# Autodesk Inventor assembly: HopperAssembly
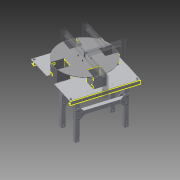
[picture p0: Inventor's stored thumbnail of the model, 180x180]
Saved by Autodesk Inventor 2013 (Build 170138000, 138)
## iProperties
Created: 2013-07-18
Part Number: HopperAssembly
Document SubType Name: Assembly
Designer: root
Author: root
## Documents named in this file (20)
- I:\FRC_Projects\Cad\Inventor_Projects\Shooter-Cleaned\HopperAssembly\HopperAssembly.iam
- I:\FRC_Projects\Cad\Inventor_Projects\Shooter-Cleaned\HopperAssembly\TopHopper\TopHopper.iam
- I:\FRC_Projects\Cad\Inventor_Projects\Shooter-Cleaned\HopperAssembly\BottomHopper\BottomHopperAssembly.iam
- I:\FRC_Projects\Cad\Inventor_Projects\Shooter-Cleaned\HopperAssembly\CouplerBridge.ipt
- I:\FRC_Projects\Cad\Inventor_Projects\Shooter-Cleaned\Libraries\ContentCenter\ANSI_ASME B18.2.1 - 1_4-20 UNC - 0.75(2).ipt
- I:\FRC_Projects\Cad\Inventor_Projects\Shooter-Cleaned\Libraries\ContentCenter\AS 2465 - 1_4  UNC(1).ipt
- I:\FRC_Projects\Cad\Inventor_Projects\Shooter-Cleaned\HopperAssembly\SpacerPvc.ipt
- I:\FRC_Projects\Cad\Inventor_Projects\Shooter-Cleaned\Libraries\ContentCenter\ANSI B18.2.2 - 1_4 - 20(2).ipt
- I:\FRC_Projects\Cad\Inventor_Projects\Shooter-Cleaned\HopperAssembly\BottomSupportBAse.ipt
- I:\FRC_Projects\Cad\Inventor_Projects\Shooter-Cleaned\HopperAssembly\BackBottonSupport.ipt
- I:\FRC_Projects\Cad\Inventor_Projects\Shooter-Cleaned\HopperAssembly\L-Bracket.ipt
- I:\FRC_Projects\Cad\Inventor_Projects\Shooter-Cleaned\Libraries\ContentCenter\ANSI_ASME B18.2.1 - 1_4-20 UNC - 1.5(2).ipt
- I:\FRC_Projects\Cad\Inventor_Projects\Shooter-Cleaned\Libraries\ContentCenter\ANSI_ASME B18.2.1 - 1_4-20 UNC - 1.75(2).ipt
- I:\FRC_Projects\Cad\Inventor_Projects\Shooter-Cleaned\HopperAssembly\TriangleBracket.ipt
- I:\FRC_Projects\Cad\Inventor_Projects\Shooter-Cleaned\HopperAssembly\BAseBAr.ipt
- I:\FRC_Projects\Cad\Inventor_Projects\Shooter-Cleaned\HopperAssembly\CrossBar.ipt
- I:\FRC_Projects\Cad\Inventor_Projects\Shooter-Cleaned\HopperAssembly\SupportT.ipt
- I:\FRC_Projects\Cad\Inventor_Projects\Shooter-Cleaned\Libraries\ContentCenter\ANSI B18.6.3 - 1_4-20 UNC - 3.25(30).ipt
- I:\FRC_Projects\Cad\Inventor_Projects\Shooter-Cleaned\HopperAssembly\TopSupportV3.ipt
- I:\FRC_Projects\Cad\Inventor_Projects\Shooter-Cleaned\Libraries\ContentCenter\ANSI B18.6.3 - 1_4-20 UNC - 2.25(30).ipt
## Components (142 placed, 19 different names)
1. BottomHopperAssembly:1 [sub-assembly] — Mate:1, Mate:2, Mate:7, Mate:11, Mate:12, Mate:13, Mate:14, Mate:111, Flush:1, Flush:2, Mate:112, Flush:3, Flush:4, Mate:113, Flush:5, Mate:183, Mate:184, Mate:185, Mate:186, Mate:187, Mate:188, Mate:189, Mate:190, Mate:258, Mate:270
2. CouplerBridge:1 — Mate:3, Mate:4, Mate:7, Mate:8, Mate:10, Mate:19, Mate:20, Mate:21, Mate:22, Mate:23, Mate:24, Mate:25, Mate:26, Mate:27, Mate:28, Mate:29, Mate:30, Mate:34, Mate:37, Mate:39, Mate:41
3. Hex Bolt - Inch 1/4-20 UNC - 0.75:1 — Mate:8, Mate:12, Mate:18
4. Hex Bolt - Inch 1/4-20 UNC - 0.75:2 — Mate:10, Mate:13, Mate:16
5. Hex Bolt - Inch 1/4-20 UNC - 0.75:3 — Mate:2, Mate:4, Mate:11, Mate:17
6. Hex Bolt - Inch 1/4-20 UNC - 0.75:4 — Mate:1, Mate:3, Mate:14, Mate:15
7. AS 2465 - Inch 1/4  UNC:1 — Mate:15, Mate:22
8. AS 2465 - Inch 1/4  UNC:2 — Mate:16, Mate:21
9. AS 2465 - Inch 1/4  UNC:3 — Mate:18, Mate:19
10. AS 2465 - Inch 1/4  UNC:4 — Mate:17, Mate:20
11. Indented Large Hex Head Machine Screw - Inch 1/4-20 UNC - 3.25:2 — Mate:23, Mate:24, Mate:40, Mate:420, Mate:427, Mate:435, Mate:456
12. Indented Large Hex Head Machine Screw - Inch 1/4-20 UNC - 3.25:3 — Mate:29, Mate:30, Mate:35, Mate:55, Mate:59, Mate:422, Mate:458
13. Indented Large Hex Head Machine Screw - Inch 1/4-20 UNC - 3.25:1 — Mate:27, Mate:28, Mate:38, Mate:425, Mate:437, Mate:452
14. Indented Large Hex Head Machine Screw - Inch 1/4-20 UNC - 3.25:4 — Mate:25, Mate:26, Mate:36, Mate:53, Mate:429, Mate:454
15. SpacerPvc:1 — Mate:36, Mate:37
16. SpacerPvc:2 — Mate:38, Mate:39
17. SpacerPvc:3 — Mate:40, Mate:41
18. SpacerPvc:4 — Mate:34, Mate:35, Mate:421
19. Hex Nut - Inch 1/4 - 20:2 — Mate:55, Mate:424
20. Hex Nut - Inch 1/4 - 20:9 — Mate:53, Mate:434
21. Hex Nut - Inch 1/4 - 20:10 — Mate:59, Mate:423
22. BottomSupportBAse:1 — Mate:112, Flush:3, Flush:4, Mate:118, Flush:7, Mate:122, Flush:9, Mate:126, Flush:11, Mate:137, Mate:138, Mate:140, Mate:145, Mate:146, Mate:147, Mate:148, Mate:149, Mate:150, Mate:192, Mate:194
23. BottomSupportBAse:2 — Mate:111, Flush:1, Flush:2, Mate:114, Flush:6, Mate:120, Flush:8, Mate:125, Mate:128, Mate:133, Mate:134, Mate:135, Mate:141, Mate:151, Mate:152, Mate:153, Mate:154, Mate:155, Mate:156, Mate:196, Mate:198, Mate:447, Flush:14
24. BackBottonSupport:2 — Mate:113, Flush:5, Mate:114, Flush:6, Mate:119, Mate:121, Mate:131, Mate:132, Mate:157, Mate:158, Mate:159, Mate:160, Mate:202, Mate:203, Mate:204, Mate:211, Mate:233, Mate:237, Mate:268, Mate:269, Mate:271, Mate:272, Mate:274, Mate:275, Mate:284, Mate:287, Mate:448
25. L-Bracket:1 — Mate:118, Mate:119, Flush:7, Mate:131, Mate:140, Mate:180, Mate:182
26. L-Bracket:2 — Mate:120, Mate:121, Flush:8, Mate:132, Mate:141, Mate:166, Mate:319
27. L-Bracket:3 — Mate:126, Flush:11, Mate:138, Mate:139, Mate:171, Mate:178
28. L-Bracket:5 — Mate:125, Mate:135, Mate:136, Mate:142, Mate:163, Mate:164, Mate:179
29. L-Bracket:6 — Mate:122, Flush:9, Mate:137, Mate:139, Mate:144, Mate:161, Mate:162, Mate:169
30. L-Bracket:7 — Mate:128, Mate:133, Mate:134, Mate:136, Mate:143, Mate:174, Mate:176
31. BackBottonSupport:3 — Mate:142, Mate:143, Mate:144, Mate:219, Mate:220, Mate:221, Mate:223, Mate:224, Mate:256, Mate:257, Mate:259, Mate:261, Mate:262, Mate:290, Mate:293
32. Hex Bolt - Inch 1/4-20 UNC - 1.5:1 — Mate:147, Mate:148, Mate:170
33. Hex Bolt - Inch 1/4-20 UNC - 1.5:2 — Mate:151, Mate:152, Mate:167
34. Hex Bolt - Inch 1/4-20 UNC - 1.5:3 — Mate:153, Mate:154, Mate:175
35. Hex Bolt - Inch 1/4-20 UNC - 1.5:4 — Mate:149, Mate:150, Mate:177
36. Hex Bolt - Inch 1/4-20 UNC - 1.5:5 — Mate:157, Mate:160, Mate:181
37. Hex Bolt - Inch 1/4-20 UNC - 1.5:6 — Mate:158, Mate:159, Mate:165
38. Hex Bolt - Inch 1/4-20 UNC - 1.5:7 — Mate:155, Mate:156, Mate:318
39. Hex Bolt - Inch 1/4-20 UNC - 1.5:8 — Mate:145, Mate:146, Mate:168
40. Hex Bolt - Inch 1/4-20 UNC - 1.75:1 — Mate:163, Mate:164, Mate:172
41. Hex Bolt - Inch 1/4-20 UNC - 1.75:2 — Mate:161, Mate:162, Mate:173
42. Hex Nut - Inch 1/4 - 20:21 — Mate:173, Mate:178
43. Hex Nut - Inch 1/4 - 20:22 — Mate:172, Mate:174
44. Hex Nut - Inch 1/4 - 20:23 — Mate:167, Mate:179
45. Hex Nut - Inch 1/4 - 20:24 — Mate:165, Mate:166
46. Hex Nut - Inch 1/4 - 20:25 — Mate:177, Mate:180
47. Hex Nut - Inch 1/4 - 20:26 — Mate:175, Mate:176
48. Hex Nut - Inch 1/4 - 20:27 — Mate:170, Mate:171
49. Hex Nut - Inch 1/4 - 20:28 — Mate:168, Mate:169
50. Hex Nut - Inch 1/4 - 20:29 — Mate:181, Mate:182
51. Hex Bolt - Inch 1/4-20 UNC - 1.75:3 — Mate:187, Mate:188, Mate:195
52. Hex Bolt - Inch 1/4-20 UNC - 1.75:4 — Mate:189, Mate:190, Mate:193
53. Hex Bolt - Inch 1/4-20 UNC - 1.75:5 — Mate:185, Mate:186, Mate:191
54. Hex Bolt - Inch 1/4-20 UNC - 1.75:6 — Mate:183, Mate:184, Mate:197
55. Hex Nut - Inch 1/4 - 20:30 — Mate:193, Mate:194
56. Hex Nut - Inch 1/4 - 20:31 — Mate:191, Mate:192
57. Hex Nut - Inch 1/4 - 20:32 — Mate:195, Mate:196
58. Hex Nut - Inch 1/4 - 20:33 — Mate:197, Mate:198
59. TriangleBracket:2 — Mate:202, Mate:203, Mate:204, Mate:209, Mate:210, Mate:234, Mate:235, Mate:236, Mate:282, Mate:283, Mate:297, Mate:298
60. TriangleBracket:3 — Mate:209, Mate:210, Mate:211, Mate:250, Mate:252, Mate:302
61. TriangleBracket:7 — Mate:219, Mate:220, Mate:221, Mate:222, Mate:231, Mate:232, Mate:288, Mate:289, Mate:306
62. TriangleBracket:8 — Mate:222, Mate:223, Mate:224, Mate:225, Mate:226, Mate:245, Mate:246, Mate:295, Mate:296
63. Hex Bolt - Inch 1/4-20 UNC - 1.75:7 — Mate:225, Mate:232, Mate:244
64. Hex Bolt - Inch 1/4-20 UNC - 1.75:8 — Mate:226, Mate:231, Mate:243
65. Hex Bolt - Inch 1/4-20 UNC - 1.75:9 — Mate:242, Mate:265, Mate:266
66. Hex Bolt - Inch 1/4-20 UNC - 1.75:10 — Mate:241, Mate:276, Mate:277
67. Hex Bolt - Inch 1/4-20 UNC - 1.75:11 — Mate:237, Mate:255, Mate:263
68. Hex Bolt - Inch 1/4-20 UNC - 1.75:12 — Mate:235, Mate:236, Mate:251
69. Hex Bolt - Inch 1/4-20 UNC - 1.75:13 — Mate:253, Mate:280, Mate:281
70. Hex Bolt - Inch 1/4-20 UNC - 1.75:14 — Mate:233, Mate:234, Mate:249
71. Hex Nut - Inch 1/4 - 20:34 — Mate:242, Mate:267
72. Hex Nut - Inch 1/4 - 20:35 — Mate:241, Mate:278
73. Hex Nut - Inch 1/4 - 20:36 — Mate:244, Mate:245
74. Hex Nut - Inch 1/4 - 20:37 — Mate:243, Mate:246
75. Hex Nut - Inch 1/4 - 20:38 — Mate:255, Mate:264
76. Hex Nut - Inch 1/4 - 20:39 — Mate:253, Mate:279
77. Hex Nut - Inch 1/4 - 20:40 — Mate:251, Mate:252
78. Hex Nut - Inch 1/4 - 20:41 — Mate:249, Mate:250
79. TriangleBracket:9 — Mate:256, Mate:257, Mate:258, Mate:259, Mate:260, Mate:264, Mate:265, Mate:267, Mate:307
80. TriangleBracket:10 — Mate:260, Mate:261, Mate:262, Mate:263, Mate:266, Mate:291, Mate:292, Mate:309
81. TriangleBracket:11 — Mate:268, Mate:269, Mate:270, Mate:271, Mate:273, Mate:278, Mate:279, Mate:304
82. TriangleBracket:12 — Mate:272, Mate:273, Mate:274, Mate:275, Mate:276, Mate:277, Mate:280, Mate:281, Mate:285, Mate:286, Mate:299, Mate:300
83. BAseBAr:1 — Mate:288, Mate:289, Mate:290, Mate:340, Mate:341, Mate:342, Mate:346, Mate:347, Mate:348
84. BAseBAr:2 — Mate:291, Mate:292, Mate:293, Mate:294, Flush:12, Mate:320, Mate:322, Mate:323, Mate:324, Mate:335, Mate:336
85. BAseBAr:3 — Mate:285, Mate:286, Mate:287, Flush:13, Mate:326, Mate:327, Mate:328, Mate:331, Mate:332
86. BAseBAr:4 — Mate:282, Mate:283, Mate:284, Mate:337, Mate:338, Mate:339, Mate:352, Mate:353
87. Hex Bolt - Inch 1/4-20 UNC - 1.5:9 — Mate:299, Mate:300, Mate:303
88. Hex Bolt - Inch 1/4-20 UNC - 1.5:10 — Mate:295, Mate:296, Mate:305
89. Hex Bolt - Inch 1/4-20 UNC - 1.5:11 — Mate:297, Mate:298, Mate:301
90. Hex Bolt - Inch 1/4-20 UNC - 1.5:12 — Mate:294, Mate:307, Mate:308
91. Hex Nut - Inch 1/4 - 20:42 — Mate:301, Mate:302
92. Hex Nut - Inch 1/4 - 20:43 — Mate:303, Mate:304
93. Hex Nut - Inch 1/4 - 20:44 — Mate:305, Mate:306
94. Hex Nut - Inch 1/4 - 20:45 — Mate:308, Mate:309
95. Hex Nut - Inch 1/4 - 20:47 — Mate:318, Mate:319
96. CrossBar:1 — Flush:12, Mate:320, Flush:13, Mate:321, Mate:325, Mate:329, Mate:330, Mate:333, Mate:334
97. SupportT:1 — Mate:321, Mate:322, Mate:323, Mate:324, Mate:354, Mate:355, Mate:356, Mate:360, Mate:361, Mate:362
98. SupportT:2 — Mate:329, Mate:330, Mate:331, Mate:332, Mate:393, Mate:394, Mate:395
99. SupportT:3 — Mate:325, Mate:326, Mate:327, Mate:328, Mate:357, Mate:358, Mate:359, Mate:363, Mate:364, Mate:365
100. SupportT:4 — Mate:333, Mate:334, Mate:335, Mate:336, Mate:397, Mate:399, Mate:401
101. CrossBar:2 — Mate:343, Mate:344, Mate:345, Mate:349, Mate:350, Mate:351
102. SupportT:5 — Mate:340, Mate:341, Mate:342, Mate:343, Mate:369, Mate:370, Mate:371, Mate:375, Mate:376, Mate:377
103. SupportT:6 — Mate:350, Mate:351, Mate:352, Mate:353, Mate:387, Mate:388, Mate:389
104. SupportT:7 — Mate:346, Mate:347, Mate:348, Mate:349, Mate:381, Mate:382, Mate:383
105. SupportT:8 — Mate:337, Mate:338, Mate:339, Mate:344, Mate:345, Mate:366, Mate:367, Mate:368, Mate:372, Mate:373, Mate:374
106. Hex Bolt - Inch 1/4-20 UNC - 1.75:15 — Mate:354, Mate:360, Mate:396
107. Hex Bolt - Inch 1/4-20 UNC - 1.75:16 — Mate:355, Mate:362, Mate:398
108. Hex Bolt - Inch 1/4-20 UNC - 1.75:17 — Mate:356, Mate:361, Mate:400
109. Hex Bolt - Inch 1/4-20 UNC - 1.75:18 — Mate:357, Mate:363, Mate:392
110. Hex Bolt - Inch 1/4-20 UNC - 1.75:22 — Mate:359, Mate:365, Mate:391
111. Hex Bolt - Inch 1/4-20 UNC - 1.75:23 — Mate:358, Mate:364, Mate:390
112. Hex Bolt - Inch 1/4-20 UNC - 1.75:24 — Mate:370, Mate:376, Mate:379
113. Hex Bolt - Inch 1/4-20 UNC - 1.75:25 — Mate:368, Mate:374, Mate:386
114. Hex Bolt - Inch 1/4-20 UNC - 1.75:26 — Mate:367, Mate:373, Mate:385
115. Hex Bolt - Inch 1/4-20 UNC - 1.75:27 — Mate:366, Mate:372, Mate:384
116. Hex Bolt - Inch 1/4-20 UNC - 1.75:28 — Mate:371, Mate:377, Mate:378
117. Hex Bolt - Inch 1/4-20 UNC - 1.75:29 — Mate:369, Mate:375, Mate:380
118. Hex Nut - Inch 1/4 - 20:48 — Mate:378, Mate:382
119. Hex Nut - Inch 1/4 - 20:49 — Mate:380, Mate:381
120. Hex Nut - Inch 1/4 - 20:50 — Mate:379, Mate:383
121. Hex Nut - Inch 1/4 - 20:51 — Mate:384, Mate:388
122. Hex Nut - Inch 1/4 - 20:52 — Mate:385, Mate:389
123. Hex Nut - Inch 1/4 - 20:53 — Mate:386, Mate:387
124. Hex Nut - Inch 1/4 - 20:54 — Mate:400, Mate:401
125. Hex Nut - Inch 1/4 - 20:55 — Mate:398, Mate:399
126. Hex Nut - Inch 1/4 - 20:56 — Mate:396, Mate:397
127. Hex Nut - Inch 1/4 - 20:57 — Mate:392, Mate:395
128. Hex Nut - Inch 1/4 - 20:58 — Mate:390, Mate:393
129. Hex Nut - Inch 1/4 - 20:59 — Mate:391, Mate:394
130. TopHopper:1 [sub-assembly] — Mate:420, Mate:421, Mate:422, Mate:423, Mate:424, Mate:426, Mate:428, Mate:430, Mate:434, Mate:436, Mate:438, Mate:453, Mate:455, Mate:457, Mate:459, Mate:460, Mate:464
131. Hex Nut - Inch 1/4 - 20:63 — Mate:425, Mate:426
132. Hex Nut - Inch 1/4 - 20:64 — Mate:427, Mate:428
133. Hex Nut - Inch 1/4 - 20:65 — Mate:429, Mate:430
134. Hex Nut - Inch 1/4 - 20:66 — Mate:435, Mate:436
135. Hex Nut - Inch 1/4 - 20:67 — Mate:437, Mate:438
136. TopSupportV3:1 — Mate:447, Mate:448, Flush:14, Mate:461, Mate:462
137. Hex Nut - Inch 1/4 - 20:68 — Mate:454, Mate:455
138. Hex Nut - Inch 1/4 - 20:69 — Mate:456, Mate:457
139. Hex Nut - Inch 1/4 - 20:70 — Mate:458, Mate:459
140. Hex Nut - Inch 1/4 - 20:71 — Mate:452, Mate:453
141. Indented Large Hex Head Machine Screw - Inch 1/4-20 UNC - 2.25:1 — Mate:460, Mate:461, Mate:462, Mate:463
142. Hex Nut - Inch 1/4 - 20:72 — Mate:463, Mate:464
## Relationships (333: Mate 320, Flush 13)
- Mate:1: BottomHopperAssembly:1 ↔ Hex Bolt - Inch 1/4-20 UNC - 0.75:4
- Mate:2: BottomHopperAssembly:1 ↔ Hex Bolt - Inch 1/4-20 UNC - 0.75:3
- Mate:3: CouplerBridge:1 ↔ Hex Bolt - Inch 1/4-20 UNC - 0.75:4
- Mate:4: CouplerBridge:1 ↔ Hex Bolt - Inch 1/4-20 UNC - 0.75:3
- Mate:7: BottomHopperAssembly:1 ↔ CouplerBridge:1
- Mate:8: CouplerBridge:1 ↔ Hex Bolt - Inch 1/4-20 UNC - 0.75:1
- Mate:10: CouplerBridge:1 ↔ Hex Bolt - Inch 1/4-20 UNC - 0.75:2
- Mate:11: BottomHopperAssembly:1 ↔ Hex Bolt - Inch 1/4-20 UNC - 0.75:3
- Mate:12: BottomHopperAssembly:1 ↔ Hex Bolt - Inch 1/4-20 UNC - 0.75:1
- Mate:13: BottomHopperAssembly:1 ↔ Hex Bolt - Inch 1/4-20 UNC - 0.75:2
- Mate:14: BottomHopperAssembly:1 ↔ Hex Bolt - Inch 1/4-20 UNC - 0.75:4
- Mate:15: Hex Bolt - Inch 1/4-20 UNC - 0.75:4 ↔ AS 2465 - Inch 1/4  UNC:1
- Mate:16: Hex Bolt - Inch 1/4-20 UNC - 0.75:2 ↔ AS 2465 - Inch 1/4  UNC:2
- Mate:17: Hex Bolt - Inch 1/4-20 UNC - 0.75:3 ↔ AS 2465 - Inch 1/4  UNC:4
- Mate:18: Hex Bolt - Inch 1/4-20 UNC - 0.75:1 ↔ AS 2465 - Inch 1/4  UNC:3
- Mate:19: CouplerBridge:1 ↔ AS 2465 - Inch 1/4  UNC:3
- Mate:20: CouplerBridge:1 ↔ AS 2465 - Inch 1/4  UNC:4
- Mate:21: CouplerBridge:1 ↔ AS 2465 - Inch 1/4  UNC:2
- Mate:22: CouplerBridge:1 ↔ AS 2465 - Inch 1/4  UNC:1
- Mate:23: CouplerBridge:1 ↔ Indented Large Hex Head Machine Screw - Inch 1/4-20 UNC - 3.25:2
- Mate:24: CouplerBridge:1 ↔ Indented Large Hex Head Machine Screw - Inch 1/4-20 UNC - 3.25:2
- Mate:26: CouplerBridge:1 ↔ Indented Large Hex Head Machine Screw - Inch 1/4-20 UNC - 3.25:4
- Mate:27: CouplerBridge:1 ↔ Indented Large Hex Head Machine Screw - Inch 1/4-20 UNC - 3.25:1
- Mate:28: CouplerBridge:1 ↔ Indented Large Hex Head Machine Screw - Inch 1/4-20 UNC - 3.25:1
- Mate:29: CouplerBridge:1 ↔ Indented Large Hex Head Machine Screw - Inch 1/4-20 UNC - 3.25:3
- Mate:30: CouplerBridge:1 ↔ Indented Large Hex Head Machine Screw - Inch 1/4-20 UNC - 3.25:3
- Mate:34: CouplerBridge:1 ↔ SpacerPvc:4
- Mate:35: Indented Large Hex Head Machine Screw - Inch 1/4-20 UNC - 3.25:3 ↔ SpacerPvc:4
- Mate:36: Indented Large Hex Head Machine Screw - Inch 1/4-20 UNC - 3.25:4 ↔ SpacerPvc:1
- Mate:37: CouplerBridge:1 ↔ SpacerPvc:1
- Mate:38: Indented Large Hex Head Machine Screw - Inch 1/4-20 UNC - 3.25:1 ↔ SpacerPvc:2
- Mate:39: CouplerBridge:1 ↔ SpacerPvc:2
- Mate:40: Indented Large Hex Head Machine Screw - Inch 1/4-20 UNC - 3.25:2 ↔ SpacerPvc:3
- Mate:41: CouplerBridge:1 ↔ SpacerPvc:3
- Mate:53: Indented Large Hex Head Machine Screw - Inch 1/4-20 UNC - 3.25:4 ↔ Hex Nut - Inch 1/4 - 20:9
- Mate:55: Indented Large Hex Head Machine Screw - Inch 1/4-20 UNC - 3.25:3 ↔ Hex Nut - Inch 1/4 - 20:2
- Mate:59: Indented Large Hex Head Machine Screw - Inch 1/4-20 UNC - 3.25:3 ↔ Hex Nut - Inch 1/4 - 20:10
- Mate:111: BottomHopperAssembly:1 ↔ BottomSupportBAse:2
- Flush:1: BottomHopperAssembly:1 ↔ BottomSupportBAse:2
- Flush:2: BottomHopperAssembly:1 ↔ BottomSupportBAse:2
- Mate:112: BottomHopperAssembly:1 ↔ BottomSupportBAse:1
- Flush:3: BottomHopperAssembly:1 ↔ BottomSupportBAse:1
- Flush:4: BottomHopperAssembly:1 ↔ BottomSupportBAse:1
- Mate:113: BottomHopperAssembly:1 ↔ BackBottonSupport:2
- Flush:5: BottomHopperAssembly:1 ↔ BackBottonSupport:2
- Mate:114: BottomSupportBAse:2 ↔ BackBottonSupport:2
- Flush:6: BottomSupportBAse:2 ↔ BackBottonSupport:2
- Mate:118: BottomSupportBAse:1 ↔ L-Bracket:1
- Mate:119: BackBottonSupport:2 ↔ L-Bracket:1
- Flush:7: BottomSupportBAse:1 ↔ L-Bracket:1
- Mate:120: BottomSupportBAse:2 ↔ L-Bracket:2
- Mate:121: BackBottonSupport:2 ↔ L-Bracket:2
- Flush:8: BottomSupportBAse:2 ↔ L-Bracket:2
- Mate:122: BottomSupportBAse:1 ↔ L-Bracket:6
- Flush:9: BottomSupportBAse:1 ↔ L-Bracket:6
- Mate:125: BottomSupportBAse:2 ↔ L-Bracket:5
- Mate:126: BottomSupportBAse:1 ↔ L-Bracket:3
- Flush:11: BottomSupportBAse:1 ↔ L-Bracket:3
- Mate:128: BottomSupportBAse:2 ↔ L-Bracket:7
- Mate:131: BackBottonSupport:2 ↔ L-Bracket:1
- Mate:132: BackBottonSupport:2 ↔ L-Bracket:2
- Mate:133: BottomSupportBAse:2 ↔ L-Bracket:7
- Mate:134: BottomSupportBAse:2 ↔ L-Bracket:7
- Mate:135: BottomSupportBAse:2 ↔ L-Bracket:5
- Mate:136: L-Bracket:5 ↔ L-Bracket:7
- Mate:137: BottomSupportBAse:1 ↔ L-Bracket:6
- Mate:138: BottomSupportBAse:1 ↔ L-Bracket:3
- Mate:139: L-Bracket:3 ↔ L-Bracket:6
- Mate:140: BottomSupportBAse:1 ↔ L-Bracket:1
- Mate:141: BottomSupportBAse:2 ↔ L-Bracket:2
- Mate:142: L-Bracket:5 ↔ BackBottonSupport:3
- Mate:143: L-Bracket:7 ↔ BackBottonSupport:3
- Mate:144: L-Bracket:6 ↔ BackBottonSupport:3
- Mate:145: BottomSupportBAse:1 ↔ Hex Bolt - Inch 1/4-20 UNC - 1.5:8
- Mate:146: BottomSupportBAse:1 ↔ Hex Bolt - Inch 1/4-20 UNC - 1.5:8
- Mate:147: BottomSupportBAse:1 ↔ Hex Bolt - Inch 1/4-20 UNC - 1.5:1
- Mate:148: BottomSupportBAse:1 ↔ Hex Bolt - Inch 1/4-20 UNC - 1.5:1
- Mate:149: BottomSupportBAse:1 ↔ Hex Bolt - Inch 1/4-20 UNC - 1.5:4
- Mate:150: BottomSupportBAse:1 ↔ Hex Bolt - Inch 1/4-20 UNC - 1.5:4
- Mate:151: BottomSupportBAse:2 ↔ Hex Bolt - Inch 1/4-20 UNC - 1.5:2
- Mate:152: BottomSupportBAse:2 ↔ Hex Bolt - Inch 1/4-20 UNC - 1.5:2
- Mate:153: BottomSupportBAse:2 ↔ Hex Bolt - Inch 1/4-20 UNC - 1.5:3
- Mate:154: BottomSupportBAse:2 ↔ Hex Bolt - Inch 1/4-20 UNC - 1.5:3
- Mate:155: BottomSupportBAse:2 ↔ Hex Bolt - Inch 1/4-20 UNC - 1.5:7
- Mate:156: BottomSupportBAse:2 ↔ Hex Bolt - Inch 1/4-20 UNC - 1.5:7
- Mate:157: BackBottonSupport:2 ↔ Hex Bolt - Inch 1/4-20 UNC - 1.5:5
- Mate:158: BackBottonSupport:2 ↔ Hex Bolt - Inch 1/4-20 UNC - 1.5:6
- Mate:159: BackBottonSupport:2 ↔ Hex Bolt - Inch 1/4-20 UNC - 1.5:6
- Mate:160: BackBottonSupport:2 ↔ Hex Bolt - Inch 1/4-20 UNC - 1.5:5
- Mate:161: L-Bracket:6 ↔ Hex Bolt - Inch 1/4-20 UNC - 1.75:2
- Mate:162: L-Bracket:6 ↔ Hex Bolt - Inch 1/4-20 UNC - 1.75:2
- Mate:163: L-Bracket:5 ↔ Hex Bolt - Inch 1/4-20 UNC - 1.75:1
- Mate:164: L-Bracket:5 ↔ Hex Bolt - Inch 1/4-20 UNC - 1.75:1
- Mate:165: Hex Bolt - Inch 1/4-20 UNC - 1.5:6 ↔ Hex Nut - Inch 1/4 - 20:24
- Mate:166: L-Bracket:2 ↔ Hex Nut - Inch 1/4 - 20:24
- Mate:167: Hex Bolt - Inch 1/4-20 UNC - 1.5:2 ↔ Hex Nut - Inch 1/4 - 20:23
- Mate:168: Hex Bolt - Inch 1/4-20 UNC - 1.5:8 ↔ Hex Nut - Inch 1/4 - 20:28
- Mate:169: L-Bracket:6 ↔ Hex Nut - Inch 1/4 - 20:28
- Mate:170: Hex Bolt - Inch 1/4-20 UNC - 1.5:1 ↔ Hex Nut - Inch 1/4 - 20:27
- Mate:171: L-Bracket:3 ↔ Hex Nut - Inch 1/4 - 20:27
- Mate:172: Hex Bolt - Inch 1/4-20 UNC - 1.75:1 ↔ Hex Nut - Inch 1/4 - 20:22
- Mate:173: Hex Bolt - Inch 1/4-20 UNC - 1.75:2 ↔ Hex Nut - Inch 1/4 - 20:21
- Mate:174: L-Bracket:7 ↔ Hex Nut - Inch 1/4 - 20:22
- Mate:175: Hex Bolt - Inch 1/4-20 UNC - 1.5:3 ↔ Hex Nut - Inch 1/4 - 20:26
- Mate:176: L-Bracket:7 ↔ Hex Nut - Inch 1/4 - 20:26
- Mate:177: Hex Bolt - Inch 1/4-20 UNC - 1.5:4 ↔ Hex Nut - Inch 1/4 - 20:25
- Mate:178: L-Bracket:3 ↔ Hex Nut - Inch 1/4 - 20:21
- Mate:179: L-Bracket:5 ↔ Hex Nut - Inch 1/4 - 20:23
- Mate:180: L-Bracket:1 ↔ Hex Nut - Inch 1/4 - 20:25
- Mate:181: Hex Bolt - Inch 1/4-20 UNC - 1.5:5 ↔ Hex Nut - Inch 1/4 - 20:29
- Mate:182: L-Bracket:1 ↔ Hex Nut - Inch 1/4 - 20:29
- Mate:183: BottomHopperAssembly:1 ↔ Hex Bolt - Inch 1/4-20 UNC - 1.75:6
- Mate:184: BottomHopperAssembly:1 ↔ Hex Bolt - Inch 1/4-20 UNC - 1.75:6
- Mate:185: BottomHopperAssembly:1 ↔ Hex Bolt - Inch 1/4-20 UNC - 1.75:5
- Mate:186: BottomHopperAssembly:1 ↔ Hex Bolt - Inch 1/4-20 UNC - 1.75:5
- Mate:187: BottomHopperAssembly:1 ↔ Hex Bolt - Inch 1/4-20 UNC - 1.75:3
- Mate:188: BottomHopperAssembly:1 ↔ Hex Bolt - Inch 1/4-20 UNC - 1.75:3
- Mate:189: BottomHopperAssembly:1 ↔ Hex Bolt - Inch 1/4-20 UNC - 1.75:4
- Mate:190: BottomHopperAssembly:1 ↔ Hex Bolt - Inch 1/4-20 UNC - 1.75:4
- Mate:191: Hex Bolt - Inch 1/4-20 UNC - 1.75:5 ↔ Hex Nut - Inch 1/4 - 20:31
- Mate:192: BottomSupportBAse:1 ↔ Hex Nut - Inch 1/4 - 20:31
- Mate:193: Hex Bolt - Inch 1/4-20 UNC - 1.75:4 ↔ Hex Nut - Inch 1/4 - 20:30
- Mate:194: BottomSupportBAse:1 ↔ Hex Nut - Inch 1/4 - 20:30
- Mate:195: Hex Bolt - Inch 1/4-20 UNC - 1.75:3 ↔ Hex Nut - Inch 1/4 - 20:32
- Mate:196: BottomSupportBAse:2 ↔ Hex Nut - Inch 1/4 - 20:32
- Mate:197: Hex Bolt - Inch 1/4-20 UNC - 1.75:6 ↔ Hex Nut - Inch 1/4 - 20:33
- Mate:198: BottomSupportBAse:2 ↔ Hex Nut - Inch 1/4 - 20:33
- Mate:202: BackBottonSupport:2 ↔ TriangleBracket:2
- Mate:203: BackBottonSupport:2 ↔ TriangleBracket:2
- Mate:204: BackBottonSupport:2 ↔ TriangleBracket:2
- Mate:209: TriangleBracket:2 ↔ TriangleBracket:3
- Mate:210: TriangleBracket:2 ↔ TriangleBracket:3
- Mate:211: BackBottonSupport:2 ↔ TriangleBracket:3
- Mate:219: BackBottonSupport:3 ↔ TriangleBracket:7
- Mate:220: BackBottonSupport:3 ↔ TriangleBracket:7
- Mate:221: BackBottonSupport:3 ↔ TriangleBracket:7
- Mate:222: TriangleBracket:7 ↔ TriangleBracket:8
- Mate:223: BackBottonSupport:3 ↔ TriangleBracket:8
- Mate:224: BackBottonSupport:3 ↔ TriangleBracket:8
- Mate:225: TriangleBracket:8 ↔ Hex Bolt - Inch 1/4-20 UNC - 1.75:7
- Mate:226: TriangleBracket:8 ↔ Hex Bolt - Inch 1/4-20 UNC - 1.75:8
- Mate:231: TriangleBracket:7 ↔ Hex Bolt - Inch 1/4-20 UNC - 1.75:8
- Mate:232: TriangleBracket:7 ↔ Hex Bolt - Inch 1/4-20 UNC - 1.75:7
- Mate:233: BackBottonSupport:2 ↔ Hex Bolt - Inch 1/4-20 UNC - 1.75:14
- Mate:234: TriangleBracket:2 ↔ Hex Bolt - Inch 1/4-20 UNC - 1.75:14
- Mate:235: TriangleBracket:2 ↔ Hex Bolt - Inch 1/4-20 UNC - 1.75:12
- Mate:236: TriangleBracket:2 ↔ Hex Bolt - Inch 1/4-20 UNC - 1.75:12
- Mate:237: BackBottonSupport:2 ↔ Hex Bolt - Inch 1/4-20 UNC - 1.75:11
- Mate:241: Hex Bolt - Inch 1/4-20 UNC - 1.75:10 ↔ Hex Nut - Inch 1/4 - 20:35
- Mate:242: Hex Bolt - Inch 1/4-20 UNC - 1.75:9 ↔ Hex Nut - Inch 1/4 - 20:34
- Mate:243: Hex Bolt - Inch 1/4-20 UNC - 1.75:8 ↔ Hex Nut - Inch 1/4 - 20:37
- Mate:244: Hex Bolt - Inch 1/4-20 UNC - 1.75:7 ↔ Hex Nut - Inch 1/4 - 20:36
- Mate:245: TriangleBracket:8 ↔ Hex Nut - Inch 1/4 - 20:36
- Mate:246: TriangleBracket:8 ↔ Hex Nut - Inch 1/4 - 20:37
- Mate:249: Hex Bolt - Inch 1/4-20 UNC - 1.75:14 ↔ Hex Nut - Inch 1/4 - 20:41
- Mate:250: TriangleBracket:3 ↔ Hex Nut - Inch 1/4 - 20:41
- Mate:251: Hex Bolt - Inch 1/4-20 UNC - 1.75:12 ↔ Hex Nut - Inch 1/4 - 20:40
- Mate:252: TriangleBracket:3 ↔ Hex Nut - Inch 1/4 - 20:40
- Mate:253: Hex Bolt - Inch 1/4-20 UNC - 1.75:13 ↔ Hex Nut - Inch 1/4 - 20:39
- Mate:255: Hex Bolt - Inch 1/4-20 UNC - 1.75:11 ↔ Hex Nut - Inch 1/4 - 20:38
- Mate:256: BackBottonSupport:3 ↔ TriangleBracket:9
- Mate:257: BackBottonSupport:3 ↔ TriangleBracket:9
- Mate:258: BottomHopperAssembly:1 ↔ TriangleBracket:9
- Mate:259: BackBottonSupport:3 ↔ TriangleBracket:9
- Mate:260: TriangleBracket:9 ↔ TriangleBracket:10
- Mate:261: BackBottonSupport:3 ↔ TriangleBracket:10
- Mate:262: BackBottonSupport:3 ↔ TriangleBracket:10
- Mate:263: Hex Bolt - Inch 1/4-20 UNC - 1.75:11 ↔ TriangleBracket:10
- Mate:264: Hex Nut - Inch 1/4 - 20:38 ↔ TriangleBracket:9
- Mate:265: Hex Bolt - Inch 1/4-20 UNC - 1.75:9 ↔ TriangleBracket:9
- Mate:266: Hex Bolt - Inch 1/4-20 UNC - 1.75:9 ↔ TriangleBracket:10
- Mate:267: Hex Nut - Inch 1/4 - 20:34 ↔ TriangleBracket:9
- Mate:268: BackBottonSupport:2 ↔ TriangleBracket:11
- Mate:269: BackBottonSupport:2 ↔ TriangleBracket:11
- Mate:270: BottomHopperAssembly:1 ↔ TriangleBracket:11
- Mate:271: BackBottonSupport:2 ↔ TriangleBracket:11
- Mate:272: BackBottonSupport:2 ↔ TriangleBracket:12
- Mate:273: TriangleBracket:11 ↔ TriangleBracket:12
- Mate:274: BackBottonSupport:2 ↔ TriangleBracket:12
- Mate:275: BackBottonSupport:2 ↔ TriangleBracket:12
- Mate:276: Hex Bolt - Inch 1/4-20 UNC - 1.75:10 ↔ TriangleBracket:12
- Mate:277: Hex Bolt - Inch 1/4-20 UNC - 1.75:10 ↔ TriangleBracket:12
- Mate:278: Hex Nut - Inch 1/4 - 20:35 ↔ TriangleBracket:11
- Mate:279: Hex Nut - Inch 1/4 - 20:39 ↔ TriangleBracket:11
- Mate:280: Hex Bolt - Inch 1/4-20 UNC - 1.75:13 ↔ TriangleBracket:12
- Mate:281: Hex Bolt - Inch 1/4-20 UNC - 1.75:13 ↔ TriangleBracket:12
- Mate:282: TriangleBracket:2 ↔ BAseBAr:4
- Mate:283: TriangleBracket:2 ↔ BAseBAr:4
- Mate:284: BackBottonSupport:2 ↔ BAseBAr:4
- Mate:285: TriangleBracket:12 ↔ BAseBAr:3
- Mate:286: TriangleBracket:12 ↔ BAseBAr:3
- Mate:287: BackBottonSupport:2 ↔ BAseBAr:3
- Mate:288: TriangleBracket:7 ↔ BAseBAr:1
- Mate:289: TriangleBracket:7 ↔ BAseBAr:1
- Mate:290: BackBottonSupport:3 ↔ BAseBAr:1
- Mate:291: TriangleBracket:10 ↔ BAseBAr:2
- Mate:292: TriangleBracket:10 ↔ BAseBAr:2
- Mate:293: BackBottonSupport:3 ↔ BAseBAr:2
- Mate:294: BAseBAr:2 ↔ Hex Bolt - Inch 1/4-20 UNC - 1.5:12
- Mate:295: TriangleBracket:8 ↔ Hex Bolt - Inch 1/4-20 UNC - 1.5:10
- Mate:296: TriangleBracket:8 ↔ Hex Bolt - Inch 1/4-20 UNC - 1.5:10
- Mate:297: TriangleBracket:2 ↔ Hex Bolt - Inch 1/4-20 UNC - 1.5:11
- Mate:298: TriangleBracket:2 ↔ Hex Bolt - Inch 1/4-20 UNC - 1.5:11
- Mate:299: TriangleBracket:12 ↔ Hex Bolt - Inch 1/4-20 UNC - 1.5:9
- Mate:300: TriangleBracket:12 ↔ Hex Bolt - Inch 1/4-20 UNC - 1.5:9
- Mate:301: Hex Bolt - Inch 1/4-20 UNC - 1.5:11 ↔ Hex Nut - Inch 1/4 - 20:42
- Mate:302: TriangleBracket:3 ↔ Hex Nut - Inch 1/4 - 20:42
- Mate:303: Hex Bolt - Inch 1/4-20 UNC - 1.5:9 ↔ Hex Nut - Inch 1/4 - 20:43
- Mate:304: TriangleBracket:11 ↔ Hex Nut - Inch 1/4 - 20:43
- Mate:305: Hex Bolt - Inch 1/4-20 UNC - 1.5:10 ↔ Hex Nut - Inch 1/4 - 20:44
- Mate:306: TriangleBracket:7 ↔ Hex Nut - Inch 1/4 - 20:44
- Mate:307: TriangleBracket:9 ↔ Hex Bolt - Inch 1/4-20 UNC - 1.5:12
- Mate:308: Hex Bolt - Inch 1/4-20 UNC - 1.5:12 ↔ Hex Nut - Inch 1/4 - 20:45
- Mate:309: TriangleBracket:10 ↔ Hex Nut - Inch 1/4 - 20:45
- Mate:318: Hex Bolt - Inch 1/4-20 UNC - 1.5:7 ↔ Hex Nut - Inch 1/4 - 20:47
- Mate:319: L-Bracket:2 ↔ Hex Nut - Inch 1/4 - 20:47
- Flush:12: BAseBAr:2 ↔ CrossBar:1
- Mate:320: BAseBAr:2 ↔ CrossBar:1
- Flush:13: BAseBAr:3 ↔ CrossBar:1
- Mate:321: CrossBar:1 ↔ SupportT:1
- Mate:322: BAseBAr:2 ↔ SupportT:1
- Mate:323: BAseBAr:2 ↔ SupportT:1
- Mate:324: BAseBAr:2 ↔ SupportT:1
- Mate:325: CrossBar:1 ↔ SupportT:3
- Mate:326: BAseBAr:3 ↔ SupportT:3
- Mate:327: BAseBAr:3 ↔ SupportT:3
- Mate:328: BAseBAr:3 ↔ SupportT:3
- Mate:329: CrossBar:1 ↔ SupportT:2
- Mate:330: CrossBar:1 ↔ SupportT:2
- Mate:331: BAseBAr:3 ↔ SupportT:2
- Mate:332: BAseBAr:3 ↔ SupportT:2
- Mate:333: CrossBar:1 ↔ SupportT:4
- Mate:334: CrossBar:1 ↔ SupportT:4
- Mate:335: BAseBAr:2 ↔ SupportT:4
- Mate:336: BAseBAr:2 ↔ SupportT:4
- Mate:337: BAseBAr:4 ↔ SupportT:8
- Mate:338: BAseBAr:4 ↔ SupportT:8
- Mate:339: BAseBAr:4 ↔ SupportT:8
- Mate:340: BAseBAr:1 ↔ SupportT:5
- Mate:341: BAseBAr:1 ↔ SupportT:5
- Mate:342: BAseBAr:1 ↔ SupportT:5
- Mate:343: CrossBar:2 ↔ SupportT:5
- Mate:344: CrossBar:2 ↔ SupportT:8
- Mate:345: CrossBar:2 ↔ SupportT:8
- Mate:346: BAseBAr:1 ↔ SupportT:7
- Mate:347: BAseBAr:1 ↔ SupportT:7
- Mate:348: BAseBAr:1 ↔ SupportT:7
- Mate:349: CrossBar:2 ↔ SupportT:7
- Mate:350: CrossBar:2 ↔ SupportT:6
- Mate:351: CrossBar:2 ↔ SupportT:6
- Mate:352: BAseBAr:4 ↔ SupportT:6
- Mate:353: BAseBAr:4 ↔ SupportT:6
- Mate:354: SupportT:1 ↔ Hex Bolt - Inch 1/4-20 UNC - 1.75:15
- Mate:355: SupportT:1 ↔ Hex Bolt - Inch 1/4-20 UNC - 1.75:16
- Mate:356: SupportT:1 ↔ Hex Bolt - Inch 1/4-20 UNC - 1.75:17
- Mate:357: SupportT:3 ↔ Hex Bolt - Inch 1/4-20 UNC - 1.75:18
- Mate:358: SupportT:3 ↔ Hex Bolt - Inch 1/4-20 UNC - 1.75:23
- Mate:359: SupportT:3 ↔ Hex Bolt - Inch 1/4-20 UNC - 1.75:22
- Mate:360: SupportT:1 ↔ Hex Bolt - Inch 1/4-20 UNC - 1.75:15
- Mate:361: SupportT:1 ↔ Hex Bolt - Inch 1/4-20 UNC - 1.75:17
- Mate:362: SupportT:1 ↔ Hex Bolt - Inch 1/4-20 UNC - 1.75:16
- Mate:363: SupportT:3 ↔ Hex Bolt - Inch 1/4-20 UNC - 1.75:18
- Mate:364: SupportT:3 ↔ Hex Bolt - Inch 1/4-20 UNC - 1.75:23
- Mate:365: SupportT:3 ↔ Hex Bolt - Inch 1/4-20 UNC - 1.75:22
- Mate:366: SupportT:8 ↔ Hex Bolt - Inch 1/4-20 UNC - 1.75:27
- Mate:367: SupportT:8 ↔ Hex Bolt - Inch 1/4-20 UNC - 1.75:26
- Mate:368: SupportT:8 ↔ Hex Bolt - Inch 1/4-20 UNC - 1.75:25
- Mate:369: SupportT:5 ↔ Hex Bolt - Inch 1/4-20 UNC - 1.75:29
- Mate:370: SupportT:5 ↔ Hex Bolt - Inch 1/4-20 UNC - 1.75:24
- Mate:371: SupportT:5 ↔ Hex Bolt - Inch 1/4-20 UNC - 1.75:28
- Mate:372: SupportT:8 ↔ Hex Bolt - Inch 1/4-20 UNC - 1.75:27
- Mate:373: SupportT:8 ↔ Hex Bolt - Inch 1/4-20 UNC - 1.75:26
- Mate:374: SupportT:8 ↔ Hex Bolt - Inch 1/4-20 UNC - 1.75:25
- Mate:375: SupportT:5 ↔ Hex Bolt - Inch 1/4-20 UNC - 1.75:29
- Mate:376: SupportT:5 ↔ Hex Bolt - Inch 1/4-20 UNC - 1.75:24
- Mate:377: SupportT:5 ↔ Hex Bolt - Inch 1/4-20 UNC - 1.75:28
- Mate:378: Hex Bolt - Inch 1/4-20 UNC - 1.75:28 ↔ Hex Nut - Inch 1/4 - 20:48
- Mate:379: Hex Bolt - Inch 1/4-20 UNC - 1.75:24 ↔ Hex Nut - Inch 1/4 - 20:50
- Mate:380: Hex Bolt - Inch 1/4-20 UNC - 1.75:29 ↔ Hex Nut - Inch 1/4 - 20:49
- Mate:381: SupportT:7 ↔ Hex Nut - Inch 1/4 - 20:49
- Mate:382: SupportT:7 ↔ Hex Nut - Inch 1/4 - 20:48
- Mate:383: SupportT:7 ↔ Hex Nut - Inch 1/4 - 20:50
- Mate:384: Hex Bolt - Inch 1/4-20 UNC - 1.75:27 ↔ Hex Nut - Inch 1/4 - 20:51
- Mate:385: Hex Bolt - Inch 1/4-20 UNC - 1.75:26 ↔ Hex Nut - Inch 1/4 - 20:52
- Mate:386: Hex Bolt - Inch 1/4-20 UNC - 1.75:25 ↔ Hex Nut - Inch 1/4 - 20:53
- Mate:387: SupportT:6 ↔ Hex Nut - Inch 1/4 - 20:53
- Mate:388: SupportT:6 ↔ Hex Nut - Inch 1/4 - 20:51
- Mate:389: SupportT:6 ↔ Hex Nut - Inch 1/4 - 20:52
- Mate:390: Hex Bolt - Inch 1/4-20 UNC - 1.75:23 ↔ Hex Nut - Inch 1/4 - 20:58
- Mate:391: Hex Bolt - Inch 1/4-20 UNC - 1.75:22 ↔ Hex Nut - Inch 1/4 - 20:59
- Mate:392: Hex Bolt - Inch 1/4-20 UNC - 1.75:18 ↔ Hex Nut - Inch 1/4 - 20:57
- Mate:393: SupportT:2 ↔ Hex Nut - Inch 1/4 - 20:58
- Mate:394: SupportT:2 ↔ Hex Nut - Inch 1/4 - 20:59
- Mate:395: SupportT:2 ↔ Hex Nut - Inch 1/4 - 20:57
- Mate:396: Hex Bolt - Inch 1/4-20 UNC - 1.75:15 ↔ Hex Nut - Inch 1/4 - 20:56
- Mate:397: SupportT:4 ↔ Hex Nut - Inch 1/4 - 20:56
- Mate:398: Hex Bolt - Inch 1/4-20 UNC - 1.75:16 ↔ Hex Nut - Inch 1/4 - 20:55
- Mate:399: SupportT:4 ↔ Hex Nut - Inch 1/4 - 20:55
- Mate:400: Hex Bolt - Inch 1/4-20 UNC - 1.75:17 ↔ Hex Nut - Inch 1/4 - 20:54
- Mate:401: SupportT:4 ↔ Hex Nut - Inch 1/4 - 20:54
- Mate:420: Indented Large Hex Head Machine Screw - Inch 1/4-20 UNC - 3.25:2 ↔ TopHopper:1
- Mate:421: SpacerPvc:4 ↔ TopHopper:1
- Mate:422: Indented Large Hex Head Machine Screw - Inch 1/4-20 UNC - 3.25:3 ↔ TopHopper:1
- Mate:423: Hex Nut - Inch 1/4 - 20:10 ↔ TopHopper:1
- Mate:424: Hex Nut - Inch 1/4 - 20:2 ↔ TopHopper:1
- Mate:425: Indented Large Hex Head Machine Screw - Inch 1/4-20 UNC - 3.25:1 ↔ Hex Nut - Inch 1/4 - 20:63
- Mate:426: TopHopper:1 ↔ Hex Nut - Inch 1/4 - 20:63
- Mate:427: Indented Large Hex Head Machine Screw - Inch 1/4-20 UNC - 3.25:2 ↔ Hex Nut - Inch 1/4 - 20:64
- Mate:428: TopHopper:1 ↔ Hex Nut - Inch 1/4 - 20:64
- Mate:429: Indented Large Hex Head Machine Screw - Inch 1/4-20 UNC - 3.25:4 ↔ Hex Nut - Inch 1/4 - 20:65
- Mate:430: TopHopper:1 ↔ Hex Nut - Inch 1/4 - 20:65
- Mate:434: Hex Nut - Inch 1/4 - 20:9 ↔ TopHopper:1
- Mate:435: Indented Large Hex Head Machine Screw - Inch 1/4-20 UNC - 3.25:2 ↔ Hex Nut - Inch 1/4 - 20:66
- Mate:436: TopHopper:1 ↔ Hex Nut - Inch 1/4 - 20:66
- Mate:437: Indented Large Hex Head Machine Screw - Inch 1/4-20 UNC - 3.25:1 ↔ Hex Nut - Inch 1/4 - 20:67
- Mate:438: TopHopper:1 ↔ Hex Nut - Inch 1/4 - 20:67
- Mate:447: BottomSupportBAse:2 ↔ TopSupportV3:1
- Mate:448: BackBottonSupport:2 ↔ TopSupportV3:1
- Flush:14: BottomSupportBAse:2 ↔ TopSupportV3:1
- Mate:452: Indented Large Hex Head Machine Screw - Inch 1/4-20 UNC - 3.25:1 ↔ Hex Nut - Inch 1/4 - 20:71
- Mate:453: TopHopper:1 ↔ Hex Nut - Inch 1/4 - 20:71
- Mate:454: Indented Large Hex Head Machine Screw - Inch 1/4-20 UNC - 3.25:4 ↔ Hex Nut - Inch 1/4 - 20:68
- Mate:455: TopHopper:1 ↔ Hex Nut - Inch 1/4 - 20:68
- Mate:456: Indented Large Hex Head Machine Screw - Inch 1/4-20 UNC - 3.25:2 ↔ Hex Nut - Inch 1/4 - 20:69
- Mate:457: TopHopper:1 ↔ Hex Nut - Inch 1/4 - 20:69
- Mate:458: Indented Large Hex Head Machine Screw - Inch 1/4-20 UNC - 3.25:3 ↔ Hex Nut - Inch 1/4 - 20:70
- Mate:459: TopHopper:1 ↔ Hex Nut - Inch 1/4 - 20:70
- Mate:460: TopHopper:1 ↔ Indented Large Hex Head Machine Screw - Inch 1/4-20 UNC - 2.25:1
- Mate:461: TopSupportV3:1 ↔ Indented Large Hex Head Machine Screw - Inch 1/4-20 UNC - 2.25:1
- Mate:462: TopSupportV3:1 ↔ Indented Large Hex Head Machine Screw - Inch 1/4-20 UNC - 2.25:1
- Mate:463: Indented Large Hex Head Machine Screw - Inch 1/4-20 UNC - 2.25:1 ↔ Hex Nut - Inch 1/4 - 20:72
- Mate:464: TopHopper:1 ↔ Hex Nut - Inch 1/4 - 20:72
- Mate:25: CouplerBridge:1 ↔ Indented Large Hex Head Machine Screw - Inch 1/4-20 UNC - 3.25:4
